# Autodesk Inventor assembly: pencil_assembly
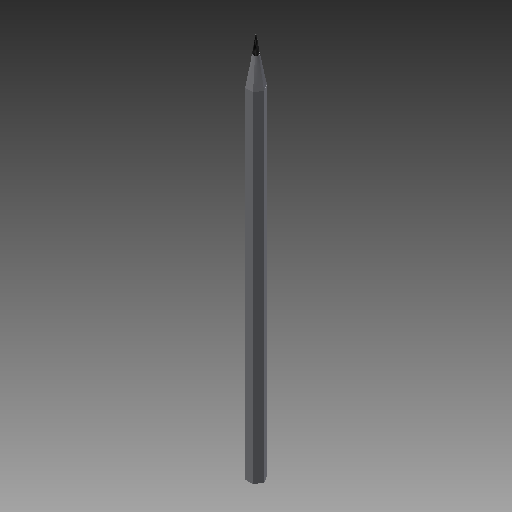
[picture p0: Inventor's stored thumbnail of the model, 512x512]
Saved by Autodesk Inventor 2017 (Build 210142000, 142)
## iProperties
Created: 2015-08-30
Part Number: pencil_assembly
Document SubType Name: Assembly
## Documents named in this file (5)
- C:\Users\Parshant Bombhi\sfuvault\Rembrant Robotics\Parshant Files\Pencil\pencil_assembly.iam
- C:\Users\Parshant Bombhi\sfuvault\Rembrant Robotics\Parshant Files\Pencil\Pencil Outside.ipt
- C:\Users\Parshant Bombhi\sfuvault\Rembrant Robotics\Parshant Files\Pencil\Pencil Shell.ipt
- C:\Users\Parshant Bombhi\sfuvault\Rembrant Robotics\Parshant Files\Pencil\Pencil Tip.ipt
- C:\Users\Parshant Bombhi\sfuvault\Rembrant Robotics\Parshant Files\Pencil\Pencil Tip 2.ipt
## Components (4 placed, 4 different names)
1. Pencil Outside:1 — Mate:1, Mate:2, Mate:3
2. Pencil Shell:1 — Mate:1, Mate:2, Mate:3, Insert:1, Insert:2
3. Pencil Tip:1 — Insert:1
4. Pencil Tip 2:1 — Insert:2
## Relationships (5: Mate 3, Insert 2)
- Mate:1: Pencil Outside:1 ↔ Pencil Shell:1
- Mate:2: Pencil Outside:1 ↔ Pencil Shell:1
- Mate:3: Pencil Outside:1 ↔ Pencil Shell:1
- Insert:1 (-10 mm): Pencil Shell:1 ↔ Pencil Tip:1
- Insert:2 (-10 mm): Pencil Shell:1 ↔ Pencil Tip 2:1
